# Autodesk Inventor assembly: Micromouse 2019 (14HM11)
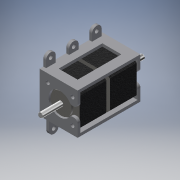
[picture p0: Inventor's stored thumbnail of the model, 180x180]
Saved by Autodesk Inventor 2019 (Build 230136000, 136)
## iProperties
Created: 2018-11-13
Part Number: Micromouse 2019 (14HM11)
Document SubType Name: Assembly
Designer: Billy
Author: Billy
## Documents named in this file (3)
- C:\Users\billy_000\Documents\Micromouse\2019\CAD\Micromouse 2019 (14HM11).iam
- C:\Users\billy_000\Documents\Micromouse\2019\CAD\14HM11 Chassis.ipt
- C:\Users\billy_000\Documents\Micromouse\2019\CAD\14HM11.ipt
## Components (3 placed, 2 different names)
1. 14HM11 Chassis:1 — Insert:1, Insert:2, Insert:3, Insert:4
2. 14HM11:1 — Insert:3, Insert:4
3. 14HM11:2 — Insert:1, Insert:2
## Relationships (4: Insert 4)
- Insert:1: 14HM11 Chassis:1 ↔ 14HM11:2
- Insert:2: 14HM11 Chassis:1 ↔ 14HM11:2
- Insert:3: 14HM11 Chassis:1 ↔ 14HM11:1
- Insert:4: 14HM11 Chassis:1 ↔ 14HM11:1
